# Autodesk Inventor assembly: DornaAI_gripper_v1
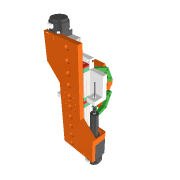
[picture p0: Inventor's stored thumbnail of the model, 180x180]
Saved by Autodesk Inventor 2022 (Build 260153000, 153)
## iProperties
Created: 2023-01-05
Part Number: DornaAI_gripper_v1
Document SubType Name: Assembly
Designer: diederichbenedict
Author: diederichbenedict
## Documents named in this file (9)
- C:\Users\diederichbenedict\Documents\Inventor\DORNA\INVENTOR\DornaAI_gripper_v1.iam
- C:\Users\diederichbenedict\Documents\Inventor\DORNA\INVENTOR\00_MGN12H, LINEAR Rail.ipt
- C:\Users\diederichbenedict\Documents\Inventor\DORNA\INVENTOR\00_MGN12H, LINEAR GUIDE BLOCK.ipt
- C:\Users\diederichbenedict\Documents\Inventor\DORNA\INVENTOR\00_Joy-IT-B20SHD4353_NEMA8_captive.ipt
- C:\Users\diederichbenedict\Documents\Inventor\DORNA\INVENTOR\dorna_2_CAD.ipt
- C:\Users\diederichbenedict\Documents\Inventor\DORNA\INVENTOR\Gripper_linear_base.ipt
- C:\Users\diederichbenedict\Documents\Inventor\DORNA\INVENTOR\Gripper_linear_arm_1.ipt
- C:\Users\diederichbenedict\Documents\Inventor\DORNA\INVENTOR\Gripper_linear_finger.ipt
- C:\Users\diederichbenedict\Documents\Inventor\DORNA\INVENTOR\Gripper_linear_finger_long.ipt
## Components (13 placed, 8 different names)
1. 00_MGN12H, LINEAR Rail:1 — Fluchtend:1, Passend:1, Passend:2, Passend:3, Fluchtend:4, Fluchtend:7, Passend:4, Passend:5, Winkel:1, Passend:6, Fluchtend:13, Passend:7
2. 00_MGN12H, LINEAR GUIDE BLOCK:1 — Passend:2, Fluchtend:2, Fluchtend:13, Fluchtend:14, Fluchtend:15
3. 00_Joy-IT-B20SHD4353_NEMA8_captive:1 — Fluchtend:4, Passend:6, Fluchtend:10, Fluchtend:12
4. 00_MGN12H, LINEAR GUIDE BLOCK:2 — Fluchtend:1, Passend:1, Fluchtend:2, Passend:7, Einfügen:1, Winkel:2
5. 00_Joy-IT-B20SHD4353_NEMA8_captive:2 — Passend:3, Fluchtend:7, Fluchtend:11
6. dorna_2_CAD:1 — Passend:4, Passend:5, Winkel:1, Fluchtend:8, Fluchtend:9
7. Gripper_linear_base:1 — Fluchtend:8, Fluchtend:9, Fluchtend:10, Fluchtend:11, Fluchtend:12
8. Gripper_linear_arm_1:1 — Fluchtend:14, Fluchtend:15, Fluchtend:16, Fluchtend:17
9. Gripper_linear_arm_1:2 — Einfügen:1, Winkel:2, Einfügen:2, Winkel:3
10. Gripper_linear_finger:1 — Fluchtend:16, Fluchtend:17, Einfügen:3
11. Gripper_linear_finger:2 — Einfügen:2, Winkel:3, Fluchtend:18, Fluchtend:19
12. Gripper_linear_finger_long:1 — Fluchtend:18, Fluchtend:19
13. Gripper_linear_finger_long:2 — Einfügen:3
## Relationships (29: Flush 16, Mate 7, Angle 3, Insert 3)
- Fluchtend:1 [Flush]: 00_MGN12H, LINEAR Rail:1 ↔ 00_MGN12H, LINEAR GUIDE BLOCK:2
- Passend:1 [Mate] (0.3 mm): 00_MGN12H, LINEAR Rail:1 ↔ 00_MGN12H, LINEAR GUIDE BLOCK:2
- Passend:2 [Mate] (0.3 mm): 00_MGN12H, LINEAR Rail:1 ↔ 00_MGN12H, LINEAR GUIDE BLOCK:1
- Fluchtend:2 [Flush]: 00_MGN12H, LINEAR GUIDE BLOCK:1 ↔ 00_MGN12H, LINEAR GUIDE BLOCK:2
- Passend:3 [Mate] (10 mm): 00_MGN12H, LINEAR Rail:1 ↔ 00_Joy-IT-B20SHD4353_NEMA8_captive:2
- Fluchtend:4 [Flush]: 00_MGN12H, LINEAR Rail:1 ↔ 00_Joy-IT-B20SHD4353_NEMA8_captive:1
- Fluchtend:7 [Flush]: 00_MGN12H, LINEAR Rail:1 ↔ 00_Joy-IT-B20SHD4353_NEMA8_captive:2
- Passend:4 [Mate] (6 mm): 00_MGN12H, LINEAR Rail:1 ↔ dorna_2_CAD:1
- Passend:5 [Mate]: 00_MGN12H, LINEAR Rail:1 ↔ dorna_2_CAD:1
- Winkel:1 [Angle] (0 deg): 00_MGN12H, LINEAR Rail:1 ↔ dorna_2_CAD:1
- Fluchtend:8 [Flush]: dorna_2_CAD:1 ↔ Gripper_linear_base:1
- Fluchtend:9 [Flush]: dorna_2_CAD:1 ↔ Gripper_linear_base:1
- Passend:6 [Mate] (10 mm): 00_MGN12H, LINEAR Rail:1 ↔ 00_Joy-IT-B20SHD4353_NEMA8_captive:1
- Fluchtend:10 [Flush] (-3 mm): 00_Joy-IT-B20SHD4353_NEMA8_captive:1 ↔ Gripper_linear_base:1
- Fluchtend:11 [Flush] (3 mm): 00_Joy-IT-B20SHD4353_NEMA8_captive:2 ↔ Gripper_linear_base:1
- Fluchtend:12 [Flush]: 00_Joy-IT-B20SHD4353_NEMA8_captive:1 ↔ Gripper_linear_base:1
- Fluchtend:13 [Flush] (0.5 mm): 00_MGN12H, LINEAR Rail:1 ↔ 00_MGN12H, LINEAR GUIDE BLOCK:1
- Passend:7 [Mate] (0.5 mm): 00_MGN12H, LINEAR Rail:1 ↔ 00_MGN12H, LINEAR GUIDE BLOCK:2
- Fluchtend:14 [Flush]: 00_MGN12H, LINEAR GUIDE BLOCK:1 ↔ Gripper_linear_arm_1:1
- Fluchtend:15 [Flush]: 00_MGN12H, LINEAR GUIDE BLOCK:1 ↔ Gripper_linear_arm_1:1
- Einfügen:1 [Insert]: 00_MGN12H, LINEAR GUIDE BLOCK:2 ↔ Gripper_linear_arm_1:2
- Winkel:2 [Angle] (0 deg): 00_MGN12H, LINEAR GUIDE BLOCK:2 ↔ Gripper_linear_arm_1:2
- Fluchtend:16 [Flush]: Gripper_linear_arm_1:1 ↔ Gripper_linear_finger:1
- Fluchtend:17 [Flush]: Gripper_linear_arm_1:1 ↔ Gripper_linear_finger:1
- Einfügen:2 [Insert]: Gripper_linear_arm_1:2 ↔ Gripper_linear_finger:2
- Winkel:3 [Angle] (0 deg): Gripper_linear_arm_1:2 ↔ Gripper_linear_finger:2
- Fluchtend:18 [Flush]: Gripper_linear_finger:2 ↔ Gripper_linear_finger_long:1
- Fluchtend:19 [Flush]: Gripper_linear_finger:2 ↔ Gripper_linear_finger_long:1
- Einfügen:3 [Insert]: Gripper_linear_finger:1 ↔ Gripper_linear_finger_long:2
